# Autodesk Inventor assembly: HGR20.ipt
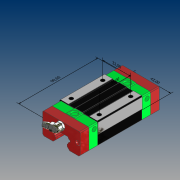
[picture p0: Inventor's stored thumbnail of the model, 180x180]
Saved by Autodesk Inventor 2021 (Build 250183000, 183)
## iProperties
Created: 2021-09-26
Part Number: HGR20.ipt
Document SubType Name: Assembly
Designer: 41601100
Author: 41601100
## Documents named in this file (5)
- C:\Users\Admin\Desktop\DO_AN_TOT_NGHIEP_2024\Mechanical\Design_in_3D\Library\hgr-20-1.snapshot.3\HGR20\HGR20.ipt.iam
- C:\Users\Admin\Desktop\DO_AN_TOT_NGHIEP_2024\Mechanical\Design_in_3D\Library\hgr-20-1.snapshot.3\HGR20\HGR20A.ipt
- C:\Users\Admin\Desktop\DO_AN_TOT_NGHIEP_2024\Mechanical\Design_in_3D\Library\hgr-20-1.snapshot.3\HGR20\HGR20B.ipt
- C:\Users\Admin\Desktop\DO_AN_TOT_NGHIEP_2024\Mechanical\Design_in_3D\Library\hgr-20-1.snapshot.3\HGR20\HGR20C.ipt
- C:\Users\Admin\Desktop\DO_AN_TOT_NGHIEP_2024\Mechanical\Design_in_3D\Library\hgr-20-1.snapshot.3\HGR20\HGR20D.ipt
## Components (6 placed, 4 different names)
1. HGR20A:1 — Mate:1, Mate:2, Mate:3, Mate:4, Mate:5, Mate:6, Mate:10
2. HGR20B:1 — Mate:1, Mate:2, Mate:3, Mate:11, Mate:12
3. HGR20B:2 — Mate:4, Mate:5, Mate:6, Mate:7, Mate:8, Mate:9
4. HGR20C:1 — Mate:7, Mate:8, Mate:9
5. HGR20C:3 — Mate:10, Mate:11, Mate:12, Mate:13, Mate:14
6. HGR20D:1 — Mate:13, Mate:14
## Relationships (14: Mate 14)
- Mate:1: HGR20A:1 ↔ HGR20B:1
- Mate:2: HGR20A:1 ↔ HGR20B:1
- Mate:3: HGR20A:1 ↔ HGR20B:1
- Mate:4: HGR20A:1 ↔ HGR20B:2
- Mate:5: HGR20A:1 ↔ HGR20B:2
- Mate:6: HGR20A:1 ↔ HGR20B:2
- Mate:7: HGR20B:2 ↔ HGR20C:1
- Mate:8: HGR20B:2 ↔ HGR20C:1
- Mate:9: HGR20B:2 ↔ HGR20C:1
- Mate:10: HGR20A:1 ↔ HGR20C:3
- Mate:11: HGR20B:1 ↔ HGR20C:3
- Mate:12: HGR20B:1 ↔ HGR20C:3
- Mate:13: HGR20C:3 ↔ HGR20D:1
- Mate:14: HGR20C:3 ↔ HGR20D:1
